# Autodesk Inventor assembly: main
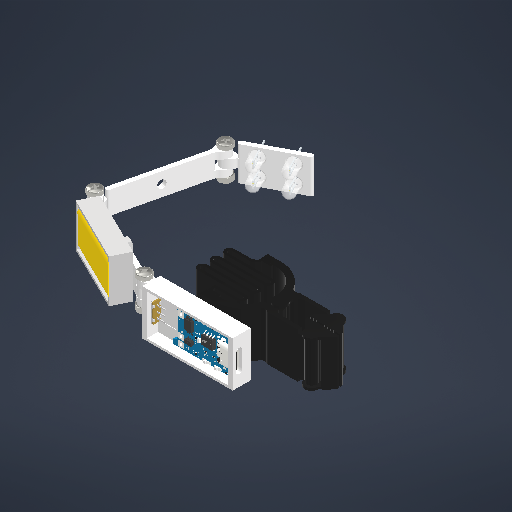
[picture p0: Inventor's stored thumbnail of the model, 512x512]
Saved by Autodesk Inventor 2027 (Build 310192060, 192F)
## iProperties
Created: 2026-05-15
Part Number: main
Document SubType Name: Assembly
Designer: User
Mass: 4.00395 g
Surface Area: 64.4201 cm^2
Volume: 4.00395 cm^3
Density: 1 g/cm^3
Author: User
## Documents named in this file (25)
- C:\Users\Duszy\Documents\Booklight\V3\main.iam
- C:\Users\Duszy\Documents\Booklight\V3\grab.ipt
- C:\Users\Duszy\Documents\Booklight\V3\arm_1.ipt
- C:\Users\Duszy\Documents\Booklight\V3\spring.ipt
- C:\Users\Duszy\Documents\Booklight\V3\arm_2.ipt
- C:\Users\Duszy\Documents\Booklight\V3\grab_MIR1.ipt
- C:\Users\Duszy\Documents\Booklight\V3\lamp_p1.ipt
- C:\Users\Duszy\Documents\Booklight\V3\lamp_link.ipt
- C:\Users\Duszy\Documents\Booklight\V3\lamp_head.ipt
- C:\Users\Duszy\Documents\Booklight\V3\elektronika.ipt
- C:\Users\Duszy\Documents\Booklight\V3\White - IR LED\White - IR LED.ipt
- C:\Users\Duszy\Documents\Booklight\V3\TP4056_Charging_Module_Type_C\TP4056_Charging_Module_Type_C.ipt
- C:\Users\Duszy\Documents\Booklight\V3\90591A250_Zinc-Plated Steel Hex Nut\90591A250_Zinc-Plated Steel Hex Nut.ipt
- C:\Users\Duszy\Documents\Booklight\V3\92005A122_Steel Pan Head Phillips Screw\92005A122_Steel Pan Head Phillips Screw.ipt
- C:\Users\Duszy\Documents\Booklight\V3\94180A331_Brass Tapered Heat-Set Inserts for Plastic\94180A331_Brass Tapered Heat-Set Inserts for Plastic.ipt
- C:\Users\Duszy\Documents\Booklight\V3\92005A114_Steel Pan Head Phillips Screw\92005A114_Steel Pan Head Phillips Screw.ipt
- C:\Users\Duszy\Documents\Booklight\V3\SPDT slide switch SS12D00\SPDT slide switch SS12D00.ipt
- C:\Users\Duszy\Documents\Booklight\V3\Battery_prop.ipt
- C:\Users\Duszy\Documents\Booklight\V3\Battery_box.ipt
- C:\Users\Duszy\Documents\Booklight\V3\main\AIP\FEA\ffhykey8w.fins
- C:\Users\Duszy\Documents\Booklight\V3\main\AIP\FEA\ffhykey9s.fsat
- C:\Users\Duszy\Documents\Booklight\V3\main\AIP\FEA\ffhykey9s.ftes
- C:\Users\Duszy\Documents\Booklight\V3\main\AIP\FEA\ffhykey9s.fwiz
- C:\Users\Duszy\Documents\Booklight\V3\main\AIP\FEA\ffhykeygw.fmsh
- C:\Users\Duszy\Documents\Booklight\V3\main\AIP\FEA\ffhykeyhs.fres
## Components (28 placed, 18 different names)
1. grab:1 — Obrotowe:5
2. arm_1:1 — Sztywne:1, Obrotowe:5
3. spring:1 — Sztywne:1, Równoległe:1, Sztywne:2
4. arm_2:1 — Sztywne:2, Obrotowe:4, Sztywne:3, Sztywne:7
5. grab_MIR1:1 — Obrotowe:4
6. lamp_p1:1 — Sztywne:3, Obrotowe:6, Obrotowe:13, Sztywne:8
7. lamp_link:1 — Obrotowe:6, Obrotowe:12, Obrotowe:14, Sztywne:9
8. lamp_head:1 — Sztywne:5, Obrotowe:15
9. elektronika:1 — Sztywne:6, Obrotowe:17, Sztywne:8, Obrotowe:18
10. TP4056_Charging_Module_Type_C:1 — Sztywne:6
11. 90591A250_Zinc-Plated Steel Hex Nut:1 — Obrotowe:8
12. 92005A122_Steel Pan Head Phillips Screw:1 — Obrotowe:8, Obrotowe:12
13. 90591A250_Zinc-Plated Steel Hex Nut:2
14. 92005A122_Steel Pan Head Phillips Screw:2 — Obrotowe:13
15. 90591A250_Zinc-Plated Steel Hex Nut:4
16. 92005A122_Steel Pan Head Phillips Screw:4 — Obrotowe:16
17. lamp_link:2 — Obrotowe:14, Obrotowe:15, Obrotowe:16
18. 94180A331_Brass Tapered Heat-Set Inserts for Plastic:1 — Sztywne:7
19. 92005A114_Steel Pan Head Phillips Screw:1 — Obrotowe:18
20. SPDT slide switch SS12D00:1 — Obrotowe:17
21. Battery_prop:1 — Obrotowe:19
22. Battery_box:1 — Sztywne:9, Obrotowe:19, Obrotowe:20
23. 92005A114_Steel Pan Head Phillips Screw:2 — Obrotowe:20, Obrotowe:21
24. 90591A250_Zinc-Plated Steel Hex Nut:5 — Obrotowe:21
25. White - IR LED:1 — Sztywne:5
26. White - IR LED:2
27. White - IR LED:3
28. White - IR LED:4
## Component patterns: (4 elements, first: White - IR LED:1)
## Relationships (25: RevoluteJoint 16, WeldJoint 8, Flush 1)
- Sztywne:1 [WeldJoint]: arm_1:1 ↔ spring:1
- Równoległe:1 [Flush] (-10 mm): spring:1
- Sztywne:2 [WeldJoint]: spring:1 ↔ arm_2:1
- Obrotowe:4 [RevoluteJoint] (0.5 mm): arm_2:1 ↔ grab_MIR1:1
- Obrotowe:5 [RevoluteJoint] (-0.5 mm): grab:1 ↔ arm_1:1
- Sztywne:3 [WeldJoint]: arm_2:1 ↔ lamp_p1:1
- Obrotowe:6 [RevoluteJoint] (0.1 mm): lamp_p1:1 ↔ lamp_link:1
- Sztywne:5 [WeldJoint]: lamp_head:1 ↔ White - IR LED:1
- Sztywne:6 [WeldJoint]: elektronika:1 ↔ TP4056_Charging_Module_Type_C:1
- Obrotowe:8 [RevoluteJoint] (-2 mm): 90591A250_Zinc-Plated Steel Hex Nut:1 ↔ 92005A122_Steel Pan Head Phillips Screw:1
- [RevoluteJoint] (-2 mm): 90591A250_Zinc-Plated Steel Hex Nut:2 ↔ 92005A122_Steel Pan Head Phillips Screw:2
- [RevoluteJoint] (-2 mm): 90591A250_Zinc-Plated Steel Hex Nut:4 ↔ 92005A122_Steel Pan Head Phillips Screw:4
- Obrotowe:12 [RevoluteJoint]: lamp_link:1 ↔ 92005A122_Steel Pan Head Phillips Screw:1
- Obrotowe:13 [RevoluteJoint]: lamp_p1:1 ↔ 92005A122_Steel Pan Head Phillips Screw:2
- Obrotowe:14 [RevoluteJoint] (-0.1 mm): lamp_link:1 ↔ lamp_link:2
- Obrotowe:15 [RevoluteJoint] (-0.1 mm): lamp_head:1 ↔ lamp_link:2
- Obrotowe:16 [RevoluteJoint]: 92005A122_Steel Pan Head Phillips Screw:4 ↔ lamp_link:2
- Sztywne:7 [WeldJoint] (3.9 mm): arm_2:1 ↔ 94180A331_Brass Tapered Heat-Set Inserts for Plastic:1
- Obrotowe:17 [RevoluteJoint]: elektronika:1 ↔ SPDT slide switch SS12D00:1
- Sztywne:8 [WeldJoint]: lamp_p1:1 ↔ elektronika:1
- Obrotowe:18 [RevoluteJoint]: elektronika:1 ↔ 92005A114_Steel Pan Head Phillips Screw:1
- Sztywne:9 [WeldJoint]: lamp_link:1 ↔ Battery_box:1
- Obrotowe:19 [RevoluteJoint]: Battery_prop:1 ↔ Battery_box:1
- Obrotowe:20 [RevoluteJoint]: Battery_box:1 ↔ 92005A114_Steel Pan Head Phillips Screw:2
- Obrotowe:21 [RevoluteJoint] (-3 mm): 92005A114_Steel Pan Head Phillips Screw:2 ↔ 90591A250_Zinc-Plated Steel Hex Nut:5
## Named parameters: sa_0 = 2000, sa_1 = 2000, d29_d25 = -2 mm, d30_d26 = -0.005051 deg, d33_d25 = -2 mm, d34_d26 = -35.946267 deg
note: some values were not read from the file. Shown as the stored number, unit unknown: "sa_0", "sa_1".
